# Autodesk Inventor assembly: VerticalSlides3.0
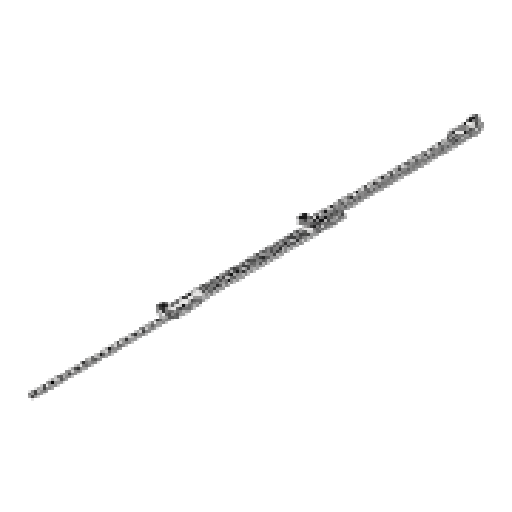
[picture p0: Inventor's stored thumbnail of the model, 512x512]
Saved by Autodesk Inventor 2023 (Build 270158000, 158)
## iProperties
Created: 2022-11-07
Part Number: VerticalSlides3.0
Document SubType Name: Assembly
Designer: deli
Author: deli
## Documents named in this file (7)
- C:\Users\deli\OneDrive - Eastside Preparatory School\FTC\8103-power-play\CAD\VerticalSlides3.0.iam
- C:\Users\deli\OneDrive - Eastside Preparatory School\FTC\8103-power-play\CAD\mgn7c carrige.ipt
- C:\Users\deli\OneDrive - Eastside Preparatory School\FTC\8103-power-play\CAD\mgn7 300mm rail.ipt
- C:\Users\deli\OneDrive - Eastside Preparatory School\FTC\8103-power-play\CAD\mgn7 300mm Connector Plate.ipt
- C:\Users\deli\OneDrive - Eastside Preparatory School\FTC\8103-power-play\CAD\mgn7SlideBearingHolder.ipt
- C:\Users\deli\OneDrive - Eastside Preparatory School\FTC\8103-power-play\CAD\mgn7SlideBearingHolder_MIR.ipt
- C:\Users\deli\OneDrive - Eastside Preparatory School\FTC\8103-power-play\CAD\Slides Bearings.iam
## Components (16 placed, 6 different names)
1. mgn7c carrige:1 — Mate:1, Mate:2, Flush:1, Mate:3, Flush:2
2. mgn7 300mm rail:1 — Mate:1, Mate:2, Flush:6
3. mgn7c carrige:2 — Flush:1, Mate:3, Flush:2, Mate:4, Mate:5, Mate:6, Flush:6
4. mgn7 300mm Connector Plate:1 — Mate:4, Mate:5, Mate:6, Mate:10, Mate:11, Mate:12, Mate:29, Mate:30, Angle:2, Mate:35, Mate:36, Angle:4
5. mgn7c carrige:3 — Mate:11, Mate:12, Flush:5
6. mgn7 300mm rail:2 — Flush:5, Mate:13, Mate:16, Mate:23, Mate:24, Mate:25, Mate:26
7. mgn7c carrige:4 — Mate:10
8. mgn7SlideBearingHolder:1 — Mate:13, Mate:22, Mate:25, Mate:26, Mate:31, Mate:32, Angle:1
9. mgn7SlideBearingHolder_MIR:1 — Mate:16, Mate:23, Mate:24, Mate:27, Mate:28, Mate:33, Mate:34
10. mgn7c carrige:5 — Angle:3
11. mgn7 300mm rail:3 — Mate:22, Mate:27, Mate:28
12. mgn7c carrige:6
13. Slides Bearings:1 [sub-assembly] — Mate:29, Mate:30, Angle:2
14. Slides Bearings:2 [sub-assembly] — Mate:31, Mate:32, Angle:1
15. Slides Bearings:3 [sub-assembly] — Mate:33, Mate:34, Angle:3
16. Slides Bearings:4 [sub-assembly] — Mate:35, Mate:36, Angle:4
## Relationships (45: Mate 32, Flush 9, Angle 4)
- Mate:1: mgn7c carrige:1 ↔ mgn7 300mm rail:1
- Mate:2: mgn7c carrige:1 ↔ mgn7 300mm rail:1
- Flush:1: mgn7c carrige:1 ↔ mgn7c carrige:2
- Mate:3: mgn7c carrige:1 ↔ mgn7c carrige:2
- Flush:2: mgn7c carrige:1 ↔ mgn7c carrige:2
- Mate:4: mgn7c carrige:2 ↔ mgn7 300mm Connector Plate:1
- Mate:5: mgn7c carrige:2 ↔ mgn7 300mm Connector Plate:1
- Mate:6: mgn7c carrige:2 ↔ mgn7 300mm Connector Plate:1
- [Mate]: mgn7c carrige:3 ↔ mgn7 300mm rail:2
- [Mate]: mgn7c carrige:3 ↔ mgn7 300mm rail:2
- [Flush]: mgn7c carrige:3 ↔ mgn7c carrige:4
- [Mate]: mgn7c carrige:3 ↔ mgn7c carrige:4
- [Flush]: mgn7c carrige:3 ↔ mgn7c carrige:4
- Mate:10: mgn7 300mm Connector Plate:1 ↔ mgn7c carrige:4
- Mate:11: mgn7 300mm Connector Plate:1 ↔ mgn7c carrige:3
- Mate:12: mgn7 300mm Connector Plate:1 ↔ mgn7c carrige:3
- Flush:5: mgn7c carrige:3 ↔ mgn7 300mm rail:2
- Flush:6: mgn7 300mm rail:1 ↔ mgn7c carrige:2
- Mate:13: mgn7 300mm rail:2 ↔ mgn7SlideBearingHolder:1
- Mate:16: mgn7 300mm rail:2 ↔ mgn7SlideBearingHolder_MIR:1
- [Mate]: mgn7c carrige:5 ↔ mgn7 300mm rail:3
- [Mate]: mgn7c carrige:5 ↔ mgn7 300mm rail:3
- [Flush]: mgn7c carrige:5 ↔ mgn7c carrige:6
- [Mate]: mgn7c carrige:5 ↔ mgn7c carrige:6
- [Flush]: mgn7c carrige:5 ↔ mgn7c carrige:6
- [Flush]: mgn7c carrige:5 ↔ mgn7 300mm rail:3
- Mate:22: mgn7SlideBearingHolder:1 ↔ mgn7 300mm rail:3
- Mate:23: mgn7 300mm rail:2 ↔ mgn7SlideBearingHolder_MIR:1
- Mate:24: mgn7 300mm rail:2 ↔ mgn7SlideBearingHolder_MIR:1
- Mate:25: mgn7 300mm rail:2 ↔ mgn7SlideBearingHolder:1
- Mate:26: mgn7 300mm rail:2 ↔ mgn7SlideBearingHolder:1
- Mate:27: mgn7SlideBearingHolder_MIR:1 ↔ mgn7 300mm rail:3
- Mate:28: mgn7SlideBearingHolder_MIR:1 ↔ mgn7 300mm rail:3
- Mate:29: mgn7 300mm Connector Plate:1 ↔ Slides Bearings:1
- Mate:30: mgn7 300mm Connector Plate:1 ↔ Slides Bearings:1
- Mate:31: mgn7SlideBearingHolder:1 ↔ Slides Bearings:2
- Mate:32: mgn7SlideBearingHolder:1 ↔ Slides Bearings:2
- Angle:1 (0 deg): mgn7SlideBearingHolder:1 ↔ Slides Bearings:2
- Angle:2 (0 deg): mgn7 300mm Connector Plate:1 ↔ Slides Bearings:1
- Mate:33: mgn7SlideBearingHolder_MIR:1 ↔ Slides Bearings:3
- Mate:34: mgn7SlideBearingHolder_MIR:1 ↔ Slides Bearings:3
- Mate:35: mgn7 300mm Connector Plate:1 ↔ Slides Bearings:4
- Mate:36: mgn7 300mm Connector Plate:1 ↔ Slides Bearings:4
- Angle:3 (0 deg): mgn7c carrige:5 ↔ Slides Bearings:3
- Angle:4 (0 deg): mgn7 300mm Connector Plate:1 ↔ Slides Bearings:4
## Named parameters: d10_d4 = 0 mm, d11_d5 = 0 mm, d12_d6 = 0 mm, d13_d2 = 0 mm, d14_d3 = 0 mm, stroke = 0 mm, d26_d10_d4 = 0 mm, d27_d11_d5 = 0 mm, d28_d12_d6 = 0 mm, d29_d13_d2 = 0 mm, d30_d14_d3 = 0 mm, d32_d18 = 0 mm
